# Autodesk Inventor assembly: Assembly
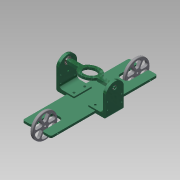
[picture p0: Inventor's stored thumbnail of the model, 180x180]
Saved by Autodesk Inventor 2019 (Build 230136000, 136)
## iProperties
Created: 2020-03-03
Part Number: Assembly
Material: Genérico
Document SubType Name: Assembly
Designer: daniel.regner
Author: daniel.regner
## Documents named in this file (7)
- \\fileserver\users\daniel.regner\Documents\Control-Gyro-stabilized-Motor-MPC\Mechanic\Inventor\V2\Assembly.iam
- \\fileserver\users\daniel.regner\Documents\Control-Gyro-stabilized-Motor-MPC\Mechanic\Inventor\V2\Chassis.ipt
- \\fileserver\users\daniel.regner\Documents\Control-Gyro-stabilized-Motor-MPC\Mechanic\Inventor\V2\Lateral support.ipt
- \\fileserver\users\daniel.regner\Documents\Control-Gyro-stabilized-Motor-MPC\Mechanic\Inventor\V2\Assembly\Design Accelerator\Rolamento4.iam
- \\fileserver\users\daniel.regner\Documents\Control-Gyro-stabilized-Motor-MPC\Mechanic\Inventor\V2\Assembly\Design Accelerator\Rolamento5.iam
- \\fileserver\users\daniel.regner\Documents\Control-Gyro-stabilized-Motor-MPC\Mechanic\Inventor\V2\Gyro support.ipt
- \\fileserver\users\daniel.regner\Documents\Control-Gyro-stabilized-Motor-MPC\Mechanic\Inventor\V2\Wheel.ipt
## Components (8 placed, 5 different names)
1. Chassis:1 — Alinhamento:1, Alinhamento:2, Alinhamento:3, Coincidência:1, Coincidência:2, Coincidência:3, Coincidência:4, Coincidência:5, Coincidência:6, Coincidência:12, Coincidência:13
2. Lateral support:1 — Coincidência:1, Coincidência:2, Coincidência:3, Coincidência:9, Coincidência:10, Coincidência:11
3. Lateral support:2 — Coincidência:4, Coincidência:5, Coincidência:6, Coincidência:7, Coincidência:8
4. Rolamento:1 [sub-assembly] — Coincidência:7, Coincidência:8
5. Rolamento:2 [sub-assembly] — Coincidência:9, Coincidência:10
6. Gyro support:1 — Coincidência:11, Alinhamento:4
7. Wheel:1 — Coincidência:12, Alinhamento:5, Alinhamento:6
8. Wheel:2 — Coincidência:13, Alinhamento:5
## Relationships (19: Mate 13, Flush 6)
- Alinhamento:1 [Flush]: Chassis:1
- Alinhamento:2 [Flush]: Chassis:1
- Alinhamento:3 [Flush]: Chassis:1
- Coincidência:1 [Mate]: Chassis:1 ↔ Lateral support:1
- Coincidência:2 [Mate]: Chassis:1 ↔ Lateral support:1
- Coincidência:3 [Mate]: Chassis:1 ↔ Lateral support:1
- Coincidência:4 [Mate]: Chassis:1 ↔ Lateral support:2
- Coincidência:5 [Mate]: Chassis:1 ↔ Lateral support:2
- Coincidência:6 [Mate]: Chassis:1 ↔ Lateral support:2
- Coincidência:7 [Mate]: Lateral support:2 ↔ Rolamento:1
- Coincidência:8 [Mate]: Lateral support:2 ↔ Rolamento:1
- Coincidência:9 [Mate]: Lateral support:1 ↔ Rolamento:2
- Coincidência:10 [Mate]: Lateral support:1 ↔ Rolamento:2
- Coincidência:11 [Mate]: Lateral support:1 ↔ Gyro support:1
- Alinhamento:4 [Flush]: Gyro support:1
- Coincidência:12 [Mate]: Chassis:1 ↔ Wheel:1
- Coincidência:13 [Mate]: Chassis:1 ↔ Wheel:2
- Alinhamento:5 [Flush]: Wheel:1 ↔ Wheel:2
- Alinhamento:6 [Flush]: Wheel:1
